# Autodesk Inventor assembly: Bed stand
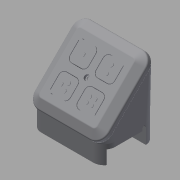
[picture p0: Inventor's stored thumbnail of the model, 180x180]
Saved by Autodesk Inventor 2020 (Build 240168000, 168)
## iProperties
Created: 2020-03-23
Part Number: Bed stand
Document SubType Name: Assembly
Designer: user
Author: user
## Documents named in this file (4)
- D:\Documents\Github\Arduino-MiLightHub_switch\3D\Bed stand.iam
- D:\Documents\Github\Arduino-MiLightHub_switch\3D\V4.2 Plate single.ipt
- D:\Documents\Github\Arduino-MiLightHub_switch\3D\V4.2 In wall.ipt
- D:\Documents\Github\Arduino-MiLightHub_switch\3D\V4 Ikea BedStand.ipt
## Components (3 placed, 3 different names)
1. V4.2 Plate single:1 — Mate:2, Angle:1, Mate:4
2. V4.2 In wall:1 — Flush:1, Mate:3
3. V4 Ikea BedStand:1 — Mate:2, Angle:1, Flush:1, Mate:3, Mate:4, Flush:2, Flush:3, Mate:5
## Relationships (8: Mate 4, Flush 3, Angle 1)
- Mate:2: V4.2 Plate single:1 ↔ V4 Ikea BedStand:1
- Angle:1 (0 deg): V4.2 Plate single:1 ↔ V4 Ikea BedStand:1
- Flush:1: V4.2 In wall:1 ↔ V4 Ikea BedStand:1
- Mate:3: V4.2 In wall:1 ↔ V4 Ikea BedStand:1
- Mate:4: V4.2 Plate single:1 ↔ V4 Ikea BedStand:1
- Flush:2: V4 Ikea BedStand:1
- Flush:3: V4 Ikea BedStand:1
- Mate:5: V4 Ikea BedStand:1
